# Autodesk Inventor assembly: Assembly
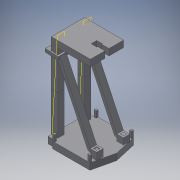
[picture p0: Inventor's stored thumbnail of the model, 180x180]
Saved by Autodesk Inventor 2016 (Build 200138000, 138)
## iProperties
Created: 2018-01-06
Part Number: Assembly
Document SubType Name: Assembly
Designer: Jorian Bruslind
Author: Jorian Bruslind
## Documents named in this file (4)
- C:\Users\Jorian Bruslind\Documents\GitHub\PersonalProjects\Inventor Projects\Maglev\Assembly.iam
- C:\Users\Jorian Bruslind\Documents\GitHub\PersonalProjects\Inventor Projects\Maglev\Maglev_Stand.ipt
- C:\Users\Jorian Bruslind\Documents\GitHub\PersonalProjects\Inventor Projects\Maglev\Maglev_supports.ipt
- C:\Users\Jorian Bruslind\Documents\GitHub\PersonalProjects\Inventor Projects\Maglev\Maglev_top.ipt
## Components (4 placed, 3 different names)
1. Maglev_Stand:1 — Mate:1, Mate:2, Mate:3, Flush:1, Mate:4, Mate:5, Flush:2, Flush:3
2. Maglev_supports:1 — Mate:1, Mate:2
3. Maglev_supports:2 — Mate:3, Flush:1, Mate:4
4. Maglev_top:1 — Mate:5, Flush:2, Flush:3
## Relationships (8: Mate 5, Flush 3)
- Mate:1: Maglev_Stand:1 ↔ Maglev_supports:1
- Mate:2: Maglev_Stand:1 ↔ Maglev_supports:1
- Mate:3: Maglev_Stand:1 ↔ Maglev_supports:2
- Flush:1: Maglev_Stand:1 ↔ Maglev_supports:2
- Mate:4: Maglev_Stand:1 ↔ Maglev_supports:2
- Mate:5: Maglev_Stand:1 ↔ Maglev_top:1
- Flush:2: Maglev_Stand:1 ↔ Maglev_top:1
- Flush:3: Maglev_Stand:1 ↔ Maglev_top:1
